# Autodesk Inventor assembly: BG001_trajan20_21
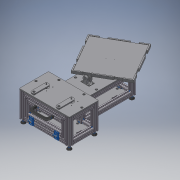
[picture p0: Inventor's stored thumbnail of the model, 180x180]
Saved by Autodesk Inventor 2022.2 (Build 262287000, 287)
## iProperties
RuleStatus: InUse
AfterDocNew0: iProperties-Editor_aufrufen
Company: HTBLA Kaindorf
Created: 2022-08-03
Part Number: BG001_trajan20_21
Project: Zeichenmaschine_v2
Material: Generisch
Description: Gerüst mit Platten
Document SubType Name: Assembly
Designer: trajan20
Author: jan
Keywords: 2021
## iProperties of the stored document 95057-030081.ipt
Created: 2022-08-03
Part Number: 95057-030081
Material: Allgemein
Description: STEP AP214
Document SubType Name: Modellieren
Designer: jan
Mass: 4.98297 g
Surface Area: 22.4459 cm^2
Volume: 4.98297 cm^3
Density: 1 g/cm^3
Appearance: Vorgabe
Company: CADENAS
Title: 95057-030081
Author: License CC BY-ND 4.0
Sending System: PARTsolutions
Preprocessor: ST-DEVELOPER v18.102
## Documents named in this file (15)
- **C:\Users\jan\Documents\DrawMachine\DrawMachineConstruction\Projekt\Zeichenmaschine_v2\BG001_trajan20_21_Zeichenmaschine_v2_Gerüst mit Platten.iam*LocalDocs*xAaaaaedaAaaaaaaaAaaaqli2Ug*95057-030081.ipt
- C:\Users\jan\Documents\DrawMachine\DrawMachineConstruction\Projekt\Zeichenmaschine_v2\BG001_trajan20_21_Zeichenmaschine_v2_Gerüst mit Platten.iam
- C:\Users\jan\Documents\DrawMachine\DrawMachineConstruction\Projekt\Zeichenmaschine_v2\BT001_trajan20_21_Zeichenmaschine_v2_Platte Stepper Motoren.ipt
- C:\Users\jan\Documents\DrawMachine\DrawMachineConstruction\Projekt\Zeichenmaschine_v2\BT002_trajan20_21_Zeichenmaschine_v2_Platte Getriebemotor.ipt
- C:\Users\jan\Documents\DrawMachine\DrawMachineConstruction\Projekt\Zeichenmaschine_v2\gerüst_v3.iam
- C:\Users\jan\Documents\DrawMachine\DrawMachineConstruction\Projekt\Zeichenmaschine_v2\importierte bauteile\Steppermotor.ipt
- C:\Users\jan\Documents\DrawMachine\DrawMachineConstruction\Projekt\Zeichenmaschine_v2\importierte bauteile\Getriebemotor.ipt
- C:\Users\jan\Documents\DrawMachine\DrawMachineConstruction\Projekt\Zeichenmaschine_v2\BT005_trajan20_21_Zeichenmaschine_v2_getriebemotor platte unten.ipt
- C:\Users\jan\Documents\DrawMachine\DrawMachineConstruction\Projekt\Zeichenmaschine_v2\BT004_trajan20_21_Zeichenmaschine_v2_Hauptplatte unten.ipt
- C:\Users\jan\Documents\DrawMachine\DrawMachineConstruction\Projekt\Zeichenmaschine_v2\BT003_trajan20_21_Zeichenmaschine_v2_zwischenteil platte gm.ipt
- C:\Users\jan\Documents\DrawMachine\DrawMachineConstruction\Projekt\Zeichenmaschine_v2\BT001_trajan20_21_Zeichenmaschine_v2_zentrierhülse platte.ipt
- C:\Users\jan\Documents\DrawMachine\DrawMachineConstruction\Projekt\Zeichenmaschine_v2\BT002_trajan20_21_Zeichenmaschine_v2_papierplatte.ipt
- C:\Users\jan\Documents\DrawMachine\DrawMachineConstruction\Projekt\Zeichenmaschine_v2\BT001_trajan20_21_Zeichenmaschine_v2_gelenk 1.ipt
- C:\Users\jan\Documents\DrawMachine\DrawMachineConstruction\Projekt\Zeichenmaschine_v2\BT101_trajan20_21_Zeichenmaschine_v2_halterung.ipt
- C:\Users\jan\Documents\DrawMachine\DrawMachineConstruction\Projekt\Zeichenmaschine_v2\step dateien\95057-030081.stp
## Components (15 placed, 13 different names)
1. BT001_trajan20_21_Zeichenmaschine_v2_Platte Stepper Motoren:1 — Fluchtend:3, Fluchtend:4, Passend:2, Passend:3, Passend:4, Passend:5, Passend:6
2. BT002_trajan20_21_Zeichenmaschine_v2_Platte Getriebemotor:1 — Fluchtend:1, Fluchtend:2, Passend:1, Passend:7, Passend:8, Passend:26, Passend:27, Passend:28
3. gerüst_v3:1 [sub-assembly] — Fluchtend:1, Fluchtend:2, Passend:1, Fluchtend:3, Fluchtend:4, Passend:2, Winkel:1, Winkel:2, Winkel:3, Passend:9, Passend:10, Passend:11, Passend:12, Passend:13, Passend:14
4. Steppermotor:1 — Passend:5, Passend:6, Winkel:2, Passend:22, Winkel:4, Passend:23
5. Steppermotor:2 — Passend:3, Winkel:1, Passend:4, Passend:24, Winkel:5, Passend:25
6. Getriebemotor:1 — Passend:7, Winkel:3, Passend:8, Passend:31, Winkel:6
7. BT005_trajan20_21_Zeichenmaschine_v2_getriebemotor platte unten:1 — Passend:9, Passend:10, Passend:11
8. BT004_trajan20_21_Zeichenmaschine_v2_Hauptplatte unten:1 — Passend:12, Passend:13, Passend:14
9. BT003_trajan20_21_Zeichenmaschine_v2_zwischenteil platte gm:1 — Passend:17, Passend:18, Passend:20, Passend:21, Passend:31, Winkel:6
10. BT001_trajan20_21_Zeichenmaschine_v2_zentrierhülse platte:1 — Passend:17, Passend:18, Passend:19
11. BT002_trajan20_21_Zeichenmaschine_v2_papierplatte:1 — Passend:19, Passend:20, Passend:21, Passend:32
12. BT001_trajan20_21_Zeichenmaschine_v2_gelenk 1:1 — Passend:22, Winkel:4, Passend:23
13. BT001_trajan20_21_Zeichenmaschine_v2_gelenk 1:2 — Passend:24, Winkel:5, Passend:25
14. BT101_trajan20_21_Zeichenmaschine_v2_halterung:1 — Passend:26, Passend:27, Passend:28, Passend:29, Passend:30
15. 95057-030081:1 — Passend:29, Passend:30, Passend:32
## Relationships (40: Mate 30, Angle 6, Flush 4)
- Fluchtend:1 [Flush]: BT002_trajan20_21_Zeichenmaschine_v2_Platte Getriebemotor:1 ↔ gerüst_v3:1
- Fluchtend:2 [Flush]: BT002_trajan20_21_Zeichenmaschine_v2_Platte Getriebemotor:1 ↔ gerüst_v3:1
- Passend:1 [Mate]: BT002_trajan20_21_Zeichenmaschine_v2_Platte Getriebemotor:1 ↔ gerüst_v3:1
- Fluchtend:3 [Flush]: BT001_trajan20_21_Zeichenmaschine_v2_Platte Stepper Motoren:1 ↔ gerüst_v3:1
- Fluchtend:4 [Flush]: BT001_trajan20_21_Zeichenmaschine_v2_Platte Stepper Motoren:1 ↔ gerüst_v3:1
- Passend:2 [Mate]: BT001_trajan20_21_Zeichenmaschine_v2_Platte Stepper Motoren:1 ↔ gerüst_v3:1
- Passend:3 [Mate]: BT001_trajan20_21_Zeichenmaschine_v2_Platte Stepper Motoren:1 ↔ Steppermotor:2
- Winkel:1 [Angle] (0 deg): gerüst_v3:1 ↔ Steppermotor:2
- Passend:4 [Mate]: BT001_trajan20_21_Zeichenmaschine_v2_Platte Stepper Motoren:1 ↔ Steppermotor:2
- Passend:5 [Mate]: BT001_trajan20_21_Zeichenmaschine_v2_Platte Stepper Motoren:1 ↔ Steppermotor:1
- Passend:6 [Mate]: BT001_trajan20_21_Zeichenmaschine_v2_Platte Stepper Motoren:1 ↔ Steppermotor:1
- Winkel:2 [Angle] (0 deg): gerüst_v3:1 ↔ Steppermotor:1
- Passend:7 [Mate]: BT002_trajan20_21_Zeichenmaschine_v2_Platte Getriebemotor:1 ↔ Getriebemotor:1
- Winkel:3 [Angle] (0 deg): gerüst_v3:1 ↔ Getriebemotor:1
- Passend:8 [Mate]: BT002_trajan20_21_Zeichenmaschine_v2_Platte Getriebemotor:1 ↔ Getriebemotor:1
- Passend:9 [Mate]: gerüst_v3:1 ↔ BT005_trajan20_21_Zeichenmaschine_v2_getriebemotor platte unten:1
- Passend:10 [Mate]: gerüst_v3:1 ↔ BT005_trajan20_21_Zeichenmaschine_v2_getriebemotor platte unten:1
- Passend:11 [Mate]: gerüst_v3:1 ↔ BT005_trajan20_21_Zeichenmaschine_v2_getriebemotor platte unten:1
- Passend:12 [Mate]: gerüst_v3:1 ↔ BT004_trajan20_21_Zeichenmaschine_v2_Hauptplatte unten:1
- Passend:13 [Mate]: gerüst_v3:1 ↔ BT004_trajan20_21_Zeichenmaschine_v2_Hauptplatte unten:1
- Passend:14 [Mate]: gerüst_v3:1 ↔ BT004_trajan20_21_Zeichenmaschine_v2_Hauptplatte unten:1
- Passend:17 [Mate]: BT003_trajan20_21_Zeichenmaschine_v2_zwischenteil platte gm:1 ↔ BT001_trajan20_21_Zeichenmaschine_v2_zentrierhülse platte:1
- Passend:18 [Mate]: BT003_trajan20_21_Zeichenmaschine_v2_zwischenteil platte gm:1 ↔ BT001_trajan20_21_Zeichenmaschine_v2_zentrierhülse platte:1
- Passend:19 [Mate]: BT001_trajan20_21_Zeichenmaschine_v2_zentrierhülse platte:1 ↔ BT002_trajan20_21_Zeichenmaschine_v2_papierplatte:1
- Passend:20 [Mate]: BT003_trajan20_21_Zeichenmaschine_v2_zwischenteil platte gm:1 ↔ BT002_trajan20_21_Zeichenmaschine_v2_papierplatte:1
- Passend:21 [Mate]: BT003_trajan20_21_Zeichenmaschine_v2_zwischenteil platte gm:1 ↔ BT002_trajan20_21_Zeichenmaschine_v2_papierplatte:1
- Passend:22 [Mate]: Steppermotor:1 ↔ BT001_trajan20_21_Zeichenmaschine_v2_gelenk 1:1
- Winkel:4 [Angle] (0 deg): Steppermotor:1 ↔ BT001_trajan20_21_Zeichenmaschine_v2_gelenk 1:1
- Passend:23 [Mate] (2 mm): Steppermotor:1 ↔ BT001_trajan20_21_Zeichenmaschine_v2_gelenk 1:1
- Passend:24 [Mate]: Steppermotor:2 ↔ BT001_trajan20_21_Zeichenmaschine_v2_gelenk 1:2
- Winkel:5 [Angle] (0 deg): Steppermotor:2 ↔ BT001_trajan20_21_Zeichenmaschine_v2_gelenk 1:2
- Passend:25 [Mate] (2 mm): Steppermotor:2 ↔ BT001_trajan20_21_Zeichenmaschine_v2_gelenk 1:2
- Passend:26 [Mate]: BT002_trajan20_21_Zeichenmaschine_v2_Platte Getriebemotor:1 ↔ BT101_trajan20_21_Zeichenmaschine_v2_halterung:1
- Passend:27 [Mate]: BT002_trajan20_21_Zeichenmaschine_v2_Platte Getriebemotor:1 ↔ BT101_trajan20_21_Zeichenmaschine_v2_halterung:1
- Passend:28 [Mate]: BT002_trajan20_21_Zeichenmaschine_v2_Platte Getriebemotor:1 ↔ BT101_trajan20_21_Zeichenmaschine_v2_halterung:1
- Passend:29 [Mate]: BT101_trajan20_21_Zeichenmaschine_v2_halterung:1 ↔ 95057-030081:1
- Passend:30 [Mate] (0.1 mm): BT101_trajan20_21_Zeichenmaschine_v2_halterung:1 ↔ 95057-030081:1
- Passend:31 [Mate]: Getriebemotor:1 ↔ BT003_trajan20_21_Zeichenmaschine_v2_zwischenteil platte gm:1
- Winkel:6 [Angle] (0 deg): Getriebemotor:1 ↔ BT003_trajan20_21_Zeichenmaschine_v2_zwischenteil platte gm:1
- Passend:32 [Mate] (15 mm): BT002_trajan20_21_Zeichenmaschine_v2_papierplatte:1 ↔ 95057-030081:1
